# Autodesk Inventor assembly: IMS-00-000_p&g
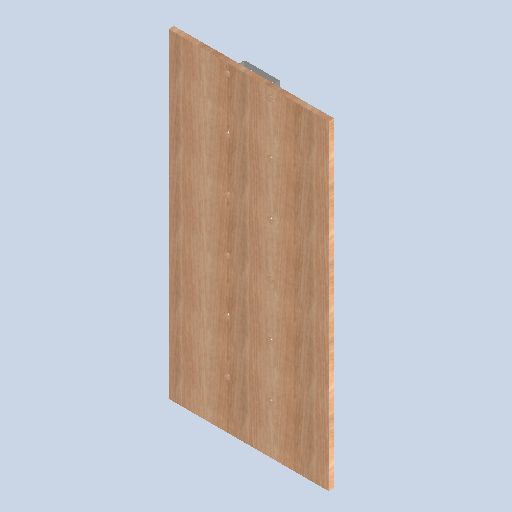
[picture p0: Inventor's stored thumbnail of the model, 512x512]
Saved by Autodesk Inventor 2025.2 (Build 292293000, 293)
## iProperties
Created: 2020-10-09
Part Number: IMS-00-000_p&g
Document SubType Name: Assembly
Designer: mahra
Author: mahra
## Documents named in this file (6)
- C:\Users\Victor\Documents\LineFollowerRobot\Anomaly_Detection\Mechanical_Project\Inventor_project\IMS-00-000_p&g.iam
- C:\Users\Victor\Documents\LineFollowerRobot\Anomaly_Detection\Mechanical_Project\Inventor_project\IMS-10-000.iam
- C:\Users\Victor\Documents\LineFollowerRobot\Anomaly_Detection\Mechanical_Project\Inventor_project\IMS-00-003.ipt
- C:\Users\mahra\Documents\Inventor\Content Center Files\R2021\en-US\DIN 7991(2)\DIN 7991 - M10x30.ipt
- C:\Users\mahra\Documents\Inventor\Content Center Files\R2021\en-US\DIN 1587\DIN 1587 - M10 x 1,5.ipt
- C:\Users\mahra\Documents\Inventor\Content Center Files\R2021\en-US\DIN 125-1  A\DIN 125 - A 10,5.ipt
## Components (32 placed, 5 different names)
1. IMS-10-000:1 [sub-assembly] — Mate:20, Flush:1
2. IMS-00-003:1 — Mate:20, Flush:1, Mate:22, Flush:2
3. DIN 1587 M10 - SW16:1
4. DIN 125-1 A A 10,5:1
5. DIN 1587 M10 - SW16:2 — Insert:5
6. DIN 125-1 A A 10,5:2 — Insert:5
7. DIN 7991 M10x30:2
8. DIN 7991 M10x30:1 — Mate:22, Flush:2
9. DIN 1587 M10 - SW16:3
10. DIN 125-1 A A 10,5:3
11. DIN 1587 M10 - SW16:4
12. DIN 125-1 A A 10,5:4
13. DIN 7991 M10x30:3
14. DIN 7991 M10x30:4
15. DIN 1587 M10 - SW16:5
16. DIN 125-1 A A 10,5:5
17. DIN 1587 M10 - SW16:6
18. DIN 125-1 A A 10,5:6
19. DIN 7991 M10x30:5
20. DIN 7991 M10x30:6
21. DIN 1587 M10 - SW16:7
22. DIN 125-1 A A 10,5:7
23. DIN 1587 M10 - SW16:8
24. DIN 125-1 A A 10,5:8
25. DIN 7991 M10x30:7
26. DIN 7991 M10x30:8
27. DIN 1587 M10 - SW16:9
28. DIN 125-1 A A 10,5:9
29. DIN 1587 M10 - SW16:10
30. DIN 125-1 A A 10,5:10
31. DIN 7991 M10x30:9
32. DIN 7991 M10x30:10
## Component patterns: (5 elements, first: DIN 1587 M10 - SW16:1 + DIN 125-1 A A 10,5:1 + DIN 1587 M10 - SW16:2 + DIN 125-1 A A 10,5:2 + DIN 7991 M10x30:2 + DIN 7991 M10x30:1)
## Relationships (7: Insert 3, Mate 2, Flush 2)
- Mate:20: IMS-10-000:1 ↔ IMS-00-003:1
- Flush:1 (10 mm): IMS-10-000:1 ↔ IMS-00-003:1
- Mate:22: IMS-00-003:1 ↔ DIN 7991 M10x30:1
- Flush:2 (1.5 mm): IMS-00-003:1 ↔ DIN 7991 M10x30:1
- [Insert]: IMS-10-000:1 ↔ DIN 125-1 A A 10,5:1
- [Insert]: DIN 1587 M10 - SW16:1 ↔ DIN 125-1 A A 10,5:1
- Insert:5: DIN 1587 M10 - SW16:2 ↔ DIN 125-1 A A 10,5:2
